# Autodesk Inventor assembly: Oreder_Alert_Counter
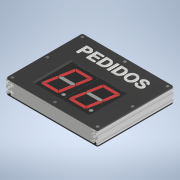
[picture p0: Inventor's stored thumbnail of the model, 180x180]
Saved by Autodesk Inventor 2020 (Build 240168000, 168)
## iProperties
Created: 2020-06-21
Part Number: Oreder_Alert_Counter
Document SubType Name: Assembly
Designer: Erick Miranda
Author: Erick Miranda
## Documents named in this file (12)
- C:\Users\Erick Miranda\Desktop\Proyectos TIA\Wi-fi Alertas de Pedidos TIA\Order_Alert_Display_Counter\3D_Model\Oreder_Alert_Counter.iam
- C:\Users\Erick Miranda\Desktop\Proyectos TIA\Wi-fi Alertas de Pedidos TIA\Order_Alert_Display_Counter\3D_Model\Display2Dig\PLDISPLAYMASTER.iam
- C:\Users\Erick Miranda\Desktop\Proyectos TIA\Wi-fi Alertas de Pedidos TIA\Order_Alert_Display_Counter\3D_Model\Back_Plate.ipt
- C:\Users\Erick Miranda\Desktop\Proyectos TIA\Wi-fi Alertas de Pedidos TIA\Order_Alert_Display_Counter\3D_Model\hexagonal_spacer_FF_M3_H10_HEX5_pass_through.ipt
- C:\Users\Erick Miranda\Desktop\Proyectos TIA\Wi-fi Alertas de Pedidos TIA\Order_Alert_Display_Counter\3D_Model\Wifi_Module\Wifi_Module.iam
- C:\Users\Erick Miranda\Desktop\Proyectos TIA\Wi-fi Alertas de Pedidos TIA\Order_Alert_Display_Counter\3D_Model\Visaton SC 4.7 ND Speaker.ipt
- C:\Users\Erick Miranda\Desktop\Proyectos TIA\Wi-fi Alertas de Pedidos TIA\Order_Alert_Display_Counter\3D_Model\73k0102_1658621-1.ipt
- C:\Users\Erick Miranda\Desktop\Proyectos TIA\Wi-fi Alertas de Pedidos TIA\Order_Alert_Display_Counter\3D_Model\Perfil20x250.ipt
- C:\Users\Erick Miranda\Desktop\Proyectos TIA\Wi-fi Alertas de Pedidos TIA\Order_Alert_Display_Counter\3D_Model\Perfil20x261.ipt
- C:\Users\Erick Miranda\Desktop\Proyectos TIA\Wi-fi Alertas de Pedidos TIA\Order_Alert_Display_Counter\3D_Model\hexagonal_spacer_FF_M3_H17_HEX5_pass_through.ipt
- C:\Users\Erick Miranda\Desktop\Proyectos TIA\Wi-fi Alertas de Pedidos TIA\Order_Alert_Display_Counter\3D_Model\Front_Plate.ipt
- C:\Users\Erick Miranda\Desktop\Proyectos TIA\Wi-fi Alertas de Pedidos TIA\Order_Alert_Display_Counter\3D_Model\TR Fastenings Ltd-M5X20mm.ipt
## Components (39 placed, 11 different names)
1. Back_Plate:1 — Rigid:12, Rotational:5, Rotational:11, Rigid:3, Rigid:4, Rigid:7, Rigid:8, Rigid:13, Rotational:13, Rotational:14, Rotational:15, Rotational:16, Rotational:17, Rotational:18, Rotational:19, Rotational:28, Rotational:29, Rotational:30, Rotational:31, Rotational:32, Rotational:33, Rotational:34, Rotational:35
2. PLDISPLAYMASTER:1 [sub-assembly] — Rigid:12, Rigid:1
3. hexagonal_spacer_FF_M3_H10_HEX5_pass_through:3 — Rotational:5
4. Wifi_Module:1 [sub-assembly] — Rigid:13, Rigid:11
5. Visaton SC 4.7 ND Speaker:1 — Rotational:11
6. 73k0102_1658621-1:1 — Rigid:1
7. 73k0102_1658621-1:2 — Rigid:11
8. Perfil20x250:1 — Rigid:3, Rigid:5
9. Perfil20x250:2 — Rigid:4, Rigid:6
10. Perfil20x250:3 — Rigid:5
11. Perfil20x250:4 — Rigid:6
12. Perfil20x261:1 — Rigid:7, Rigid:10
13. Perfil20x261:2 — Rigid:8, Rigid:9
14. Perfil20x261:3 — Rigid:9, Rigid:14
15. Perfil20x261:4 — Rigid:10
16. hexagonal_spacer_FF_M3_H10_HEX5_pass_through:4 — Rotational:13
17. hexagonal_spacer_FF_M3_H10_HEX5_pass_through:5 — Rotational:14
18. hexagonal_spacer_FF_M3_H10_HEX5_pass_through:6 — Rotational:15
19. hexagonal_spacer_FF_M3_H17_HEX5_pass_through:1 — Rotational:18
20. hexagonal_spacer_FF_M3_H17_HEX5_pass_through:2 — Rotational:16
21. hexagonal_spacer_FF_M3_H17_HEX5_pass_through:3 — Rotational:17
22. hexagonal_spacer_FF_M3_H17_HEX5_pass_through:4 — Rotational:19
23. Front_Plate:1 — Rigid:14, Rotational:20, Rotational:21, Rotational:22, Rotational:23, Rotational:24, Rotational:25, Rotational:26, Rotational:27
24. TR Fastenings Ltd-M5X20mm:1 — Rotational:23
25. TR Fastenings Ltd-M5X20mm:2 — Rotational:21
26. TR Fastenings Ltd-M5X20mm:3 — Rotational:20
27. TR Fastenings Ltd-M5X20mm:4 — Rotational:22
28. TR Fastenings Ltd-M5X20mm:5 — Rotational:24
29. TR Fastenings Ltd-M5X20mm:6 — Rotational:27
30. TR Fastenings Ltd-M5X20mm:7 — Rotational:26
31. TR Fastenings Ltd-M5X20mm:8 — Rotational:25
32. TR Fastenings Ltd-M5X20mm:9 — Rotational:28
33. TR Fastenings Ltd-M5X20mm:10 — Rotational:34
34. TR Fastenings Ltd-M5X20mm:11 — Rotational:31
35. TR Fastenings Ltd-M5X20mm:12 — Rotational:32
36. TR Fastenings Ltd-M5X20mm:13 — Rotational:30
37. TR Fastenings Ltd-M5X20mm:14 — Rotational:29
38. TR Fastenings Ltd-M5X20mm:15 — Rotational:35
39. TR Fastenings Ltd-M5X20mm:16 — Rotational:33
## Relationships (38: RevoluteJoint 25, WeldJoint 13)
- Rigid:12 [WeldJoint] (17 mm): Back_Plate:1 ↔ PLDISPLAYMASTER:1
- Rotational:5 [RevoluteJoint]: Back_Plate:1 ↔ hexagonal_spacer_FF_M3_H10_HEX5_pass_through:3
- Rotational:11 [RevoluteJoint] (9 mm): Back_Plate:1 ↔ Visaton SC 4.7 ND Speaker:1
- Rigid:1 [WeldJoint] (-4 mm): PLDISPLAYMASTER:1 ↔ 73k0102_1658621-1:1
- Rigid:3 [WeldJoint]: Back_Plate:1 ↔ Perfil20x250:1
- Rigid:4 [WeldJoint]: Back_Plate:1 ↔ Perfil20x250:2
- Rigid:5 [WeldJoint]: Perfil20x250:1 ↔ Perfil20x250:3
- Rigid:6 [WeldJoint]: Perfil20x250:2 ↔ Perfil20x250:4
- Rigid:7 [WeldJoint]: Back_Plate:1 ↔ Perfil20x261:1
- Rigid:8 [WeldJoint]: Back_Plate:1 ↔ Perfil20x261:2
- Rigid:9 [WeldJoint]: Perfil20x261:2 ↔ Perfil20x261:3
- Rigid:10 [WeldJoint]: Perfil20x261:1 ↔ Perfil20x261:4
- Rigid:13 [WeldJoint] (10 mm): Back_Plate:1 ↔ Wifi_Module:1
- Rotational:13 [RevoluteJoint]: Back_Plate:1 ↔ hexagonal_spacer_FF_M3_H10_HEX5_pass_through:4
- Rotational:14 [RevoluteJoint]: Back_Plate:1 ↔ hexagonal_spacer_FF_M3_H10_HEX5_pass_through:5
- Rotational:15 [RevoluteJoint]: Back_Plate:1 ↔ hexagonal_spacer_FF_M3_H10_HEX5_pass_through:6
- Rigid:11 [WeldJoint] (-4 mm): Wifi_Module:1 ↔ 73k0102_1658621-1:2
- Rotational:16 [RevoluteJoint]: Back_Plate:1 ↔ hexagonal_spacer_FF_M3_H17_HEX5_pass_through:2
- Rotational:17 [RevoluteJoint]: Back_Plate:1 ↔ hexagonal_spacer_FF_M3_H17_HEX5_pass_through:3
- Rotational:18 [RevoluteJoint]: Back_Plate:1 ↔ hexagonal_spacer_FF_M3_H17_HEX5_pass_through:1
- Rotational:19 [RevoluteJoint]: Back_Plate:1 ↔ hexagonal_spacer_FF_M3_H17_HEX5_pass_through:4
- Rigid:14 [WeldJoint]: Perfil20x261:3 ↔ Front_Plate:1
- Rotational:20 [RevoluteJoint]: Front_Plate:1 ↔ TR Fastenings Ltd-M5X20mm:3
- Rotational:21 [RevoluteJoint]: Front_Plate:1 ↔ TR Fastenings Ltd-M5X20mm:2
- Rotational:22 [RevoluteJoint]: Front_Plate:1 ↔ TR Fastenings Ltd-M5X20mm:4
- Rotational:23 [RevoluteJoint]: Front_Plate:1 ↔ TR Fastenings Ltd-M5X20mm:1
- Rotational:24 [RevoluteJoint]: Front_Plate:1 ↔ TR Fastenings Ltd-M5X20mm:5
- Rotational:25 [RevoluteJoint]: Front_Plate:1 ↔ TR Fastenings Ltd-M5X20mm:8
- Rotational:26 [RevoluteJoint]: Front_Plate:1 ↔ TR Fastenings Ltd-M5X20mm:7
- Rotational:27 [RevoluteJoint]: Front_Plate:1 ↔ TR Fastenings Ltd-M5X20mm:6
- Rotational:28 [RevoluteJoint]: Back_Plate:1 ↔ TR Fastenings Ltd-M5X20mm:9
- Rotational:29 [RevoluteJoint]: Back_Plate:1 ↔ TR Fastenings Ltd-M5X20mm:14
- Rotational:30 [RevoluteJoint]: Back_Plate:1 ↔ TR Fastenings Ltd-M5X20mm:13
- Rotational:31 [RevoluteJoint]: Back_Plate:1 ↔ TR Fastenings Ltd-M5X20mm:11
- Rotational:32 [RevoluteJoint]: Back_Plate:1 ↔ TR Fastenings Ltd-M5X20mm:12
- Rotational:33 [RevoluteJoint]: Back_Plate:1 ↔ TR Fastenings Ltd-M5X20mm:16
- Rotational:34 [RevoluteJoint]: Back_Plate:1 ↔ TR Fastenings Ltd-M5X20mm:10
- Rotational:35 [RevoluteJoint]: Back_Plate:1 ↔ TR Fastenings Ltd-M5X20mm:15
